# Autodesk Inventor assembly: Frame 1647030135921
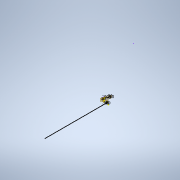
[picture p0: Inventor's stored thumbnail of the model, 180x180]
Saved by Autodesk Inventor 2022.2 (Build 262287010, 287A)
## iProperties
_FrameDoc: Frame Assembly
_Version: 25.0.0
Created: 2022-03-11
Part Number: Frame 1647030135921
Document SubType Name: Assembly
Designer: foriw
Mass: 6298.67 g
Surface Area: 9103.39 cm^2
Volume: 2238.81 cm^3
Density: 2.8134 g/cm^3
Author: foriw
## Documents named in this file (28)
- C:\Users\Finn Oriwohl\Documents\htx\1g g\BeerCart-CAD-Inventor\Workspaces\Workspace\beercart assembly - mekatronik\Frame\Frame 1647030135921.iam
- C:\Users\Finn Oriwohl\Documents\htx\1g g\BeerCart-CAD-Inventor\Workspaces\Workspace\beercart assembly - mekatronik\Frame\Skeleton 1647030135922.ipt
- C:\Users\Finn Oriwohl\Documents\htx\1g g\BeerCart-CAD-Inventor\Workspaces\Workspace\beercart assembly - mekatronik\Frame\ISO 12633-2 20x20x2 1647030639616.ipt
- C:\Users\Finn Oriwohl\Documents\htx\1g g\BeerCart-CAD-Inventor\Workspaces\Workspace\beercart assembly - mekatronik\Frame\ISO 12633-2 20x20x2 1647030639707.ipt
- C:\Users\Finn Oriwohl\Documents\htx\1g g\BeerCart-CAD-Inventor\Workspaces\Workspace\beercart assembly - mekatronik\Frame\ISO 12633-2 20x20x2 1647606177438.ipt
- C:\Users\Finn Oriwohl\Documents\htx\1g g\BeerCart-CAD-Inventor\Workspaces\Workspace\BackWheelMountingPlate.ipt
- C:\Users\Finn Oriwohl\Documents\htx\1g g\BeerCart-CAD-Inventor\Workspaces\Workspace\BackWheelMountingPlate_MIR_MIR.ipt
- C:\Users\Finn Oriwohl\Documents\htx\1g g\BeerCart-CAD-Inventor\Workspaces\Workspace\beercart assembly - mekatronik\Frame\ISO 12633-2 20x20x2 1648573909221.ipt
- C:\Users\Finn Oriwohl\Documents\htx\1g g\BeerCart-CAD-Inventor\Workspaces\Workspace\beercart assembly - mekatronik\Frame\ISO 12633-2 20x20x2 1648573975084.ipt
- C:\Users\Finn Oriwohl\Documents\htx\1g g\BeerCart-CAD-Inventor\Workspaces\Workspace\beercart assembly - mekatronik\Frame\ISO 12633-2 20x20x2 1648627088055.ipt
- C:\Users\Finn Oriwohl\Documents\htx\1g g\BeerCart-CAD-Inventor\Workspaces\Workspace\beercart assembly - mekatronik\Frame\ISO 12633-2 20x20x2 1648627088175.ipt
- C:\Users\Finn Oriwohl\Documents\htx\1g g\BeerCart-CAD-Inventor\Workspaces\Workspace\BackWheelMountingPlate_MIR4.ipt
- C:\Users\Finn Oriwohl\Documents\htx\1g g\BeerCart-CAD-Inventor\Workspaces\Workspace\beercart assembly - mekatronik\Frame\ISO 12633-2 20x20x2 1649085652950.ipt
- C:\Users\Finn Oriwohl\Documents\htx\1g g\BeerCart-CAD-Inventor\Workspaces\Workspace\beercart assembly - mekatronik\Frame\ISO 12633-2 20x20x2 1649085653040.ipt
- C:\Users\Finn Oriwohl\Documents\htx\1g g\BeerCart-CAD-Inventor\Workspaces\Workspace\backWheelNoMotor brake mount.ipt
- C:\Users\Finn Oriwohl\Documents\htx\1g g\BeerCart-CAD-Inventor\Workspaces\Workspace\beercart assembly - mekatronik\Frame\ISO 12633-2 20x20x2 1649154464355.ipt
- C:\Users\Finn Oriwohl\Documents\htx\1g g\BeerCart-CAD-Inventor\Workspaces\Workspace\BackWheelMotorMountSpacer.ipt
- C:\Users\Finn Oriwohl\Documents\htx\1g g\BeerCart-CAD-Inventor\Workspaces\Workspace\beercart assembly - mekatronik\Frame\FrontWheelFrameNew.iam
- C:\Users\Finn Oriwohl\Documents\htx\1g g\BeerCart-CAD-Inventor\Workspaces\Workspace\headset bearing.ipt
- C:\Users\Finn Oriwohl\Documents\htx\1g g\BeerCart-CAD-Inventor\Workspaces\Workspace\beercart assembly - mekatronik\Frame\ISO 12633-2 20x20x2 1650129877673.ipt
- C:\Users\Finn Oriwohl\Documents\htx\1g g\BeerCart-CAD-Inventor\Workspaces\Workspace\beercart assembly - mekatronik\Frame\ISO 12633-2 20x20x2 1650129879551.ipt
- C:\Users\Finn Oriwohl\Documents\htx\1g g\BeerCart-CAD-Inventor\Workspaces\Workspace\beercart assembly - mekatronik\Frame\ISO 12633-2 20x20x2 1650129879650.ipt
- C:\Users\Finn Oriwohl\Documents\htx\1g g\BeerCart-CAD-Inventor\Workspaces\Workspace\beercart assembly - mekatronik\Frame\ISO 12633-2 20x20x2 1650129879749.ipt
- C:\Users\Finn Oriwohl\Documents\htx\1g g\BeerCart-CAD-Inventor\Workspaces\Workspace\beercart assembly - mekatronik\Frame\ISO 12633-2 20x20x2 1650134807858.ipt
- C:\Users\Finn Oriwohl\Documents\htx\1g g\BeerCart-CAD-Inventor\Workspaces\Workspace\beercart assembly - mekatronik\Frame\plan1 .iam
- C:\Users\Finn Oriwohl\Documents\htx\1g g\BeerCart-CAD-Inventor\Workspaces\Workspace\beercart assembly - mekatronik\Frame\Plan 2 øverste.iam
- C:\Users\Finn Oriwohl\Documents\htx\1g g\BeerCart-CAD-Inventor\Workspaces\Workspace\beercart assembly - mekatronik\Frame\GlidelejrehusAssembly.iam
- C:\Users\Finn Oriwohl\Documents\htx\1g g\BeerCart-CAD-Inventor\Libraries\Content Center Files\en-US\ISO 4762(2)\ISO 4762 - M6 x 20ISO.ipt
## Components (31 placed, 23 different names)
1. Reference Skeleton
2. ISO 12633-2 20x20x2 - 250,13:1
3. ISO 12633-2 20x20x2 - 250,13:2
4. ISO 12633-2 20x20x2 - 123,73:2 — Mate:2, Mate:4, Mate:5
5. BackWheelMountingPlate:1 — Flush:6, Rotational:2, Rigid:1
6. BackWheelMountingPlate_MIR_MIR:1
7. ISO 12633-2 20x20x2 - 360,44:1
8. ISO 12633-2 20x20x2 - 105,43:1 — Flush:6, Rotational:2, Rigid:1
9. ISO 12633-2 20x20x2 - 107,97:1 — Flush:9, Flush:11, Flush:12, Flush:13, Rigid:2
10. ISO 12633-2 20x20x2 - 115.41:1
11. BackWheelMountingPlate_MIR4:1 — Flush:9, Rigid:2
12. ISO 12633-2 20x20x2 - 120.65:1 — Flush:14
13. ISO 12633-2 20x20x2 - 113,38:1 — Flush:10
14. backWheelNoMotor brake mount:1 — Flush:10, Flush:14
15. ISO 12633-2 20x20x2 - 105,43:1
16. BackWheelMotorMountSpacer:1 — Flush:11, Flush:12, Flush:13
17. FrontWheelFrameNew:1 [sub-assembly] — Insert:3, Insert:4
18. headset bearing:1 — Insert:3
19. ISO 12633-2 20x20x2 - 76,3:1
20. ISO 12633-2 20x20x2 - 85,41:1
21. ISO 12633-2 20x20x2 - 85,41:2 — Rigid:3
22. ISO 12633-2 20x20x2 - 76,3:2
23. ISO 12633-2 20x20x2 - 98,29:1
24. plan1 :1 [sub-assembly]
25. Plan 2 øverste:1 [sub-assembly]
26. GlidelejrehusAssembly:1 [sub-assembly] — Mate:20, Mate:21, Mate:22, Mate:23, Insert:4
27. GlidelejrehusAssembly:2 [sub-assembly] — Rigid:3, Mate:24, Mate:25, Mate:26, Mate:27
28. ISO 4762 M6 x 20:1 — Mate:20, Mate:21
29. ISO 4762 M6 x 20:2 — Mate:22, Mate:23
30. ISO 4762 M6 x 20:3 — Mate:24, Mate:25
31. ISO 4762 M6 x 20:4 — Mate:26, Mate:27
## Relationships (27: Mate 13, Flush 8, WeldJoint 3, Insert 2, RevoluteJoint 1)
- Mate:2: ISO 12633-2 20x20x2 - 123,73:2
- Mate:4: ISO 12633-2 20x20x2 - 123,73:2
- Mate:5: ISO 12633-2 20x20x2 - 123,73:2
- Flush:6: BackWheelMountingPlate:1 ↔ ISO 12633-2 20x20x2 - 105,43:1
- Rotational:2 [RevoluteJoint]: BackWheelMountingPlate:1 ↔ ISO 12633-2 20x20x2 - 105,43:1
- Flush:9: ISO 12633-2 20x20x2 - 107,97:1 ↔ BackWheelMountingPlate_MIR4:1
- Flush:10: ISO 12633-2 20x20x2 - 113,38:1 ↔ backWheelNoMotor brake mount:1
- Rigid:1 [WeldJoint]: BackWheelMountingPlate:1 ↔ ISO 12633-2 20x20x2 - 105,43:1
- Flush:11: ISO 12633-2 20x20x2 - 107,97:1 ↔ BackWheelMotorMountSpacer:1
- Flush:12: ISO 12633-2 20x20x2 - 107,97:1 ↔ BackWheelMotorMountSpacer:1
- Flush:13: ISO 12633-2 20x20x2 - 107,97:1 ↔ BackWheelMotorMountSpacer:1
- Flush:14: ISO 12633-2 20x20x2 - 120.65:1 ↔ backWheelNoMotor brake mount:1
- Insert:3: FrontWheelFrameNew:1 ↔ headset bearing:1
- Rigid:2 [WeldJoint]: ISO 12633-2 20x20x2 - 107,97:1 ↔ BackWheelMountingPlate_MIR4:1
- [Flush]: ISO 12633-2 20x20x2 - 85,41:1 ↔ GlidelejrehusAssembly:1
- [Mate]: FrontWheelFrameNew:1 ↔ GlidelejrehusAssembly:1
- [Mate]: ISO 12633-2 20x20x2 - 85,41:1 ↔ GlidelejrehusAssembly:1
- Rigid:3 [WeldJoint]: ISO 12633-2 20x20x2 - 85,41:2 ↔ GlidelejrehusAssembly:2
- Mate:20: GlidelejrehusAssembly:1 ↔ ISO 4762 M6 x 20:1
- Mate:21: GlidelejrehusAssembly:1 ↔ ISO 4762 M6 x 20:1
- Mate:22: GlidelejrehusAssembly:1 ↔ ISO 4762 M6 x 20:2
- Mate:23: GlidelejrehusAssembly:1 ↔ ISO 4762 M6 x 20:2
- Mate:24: GlidelejrehusAssembly:2 ↔ ISO 4762 M6 x 20:3
- Mate:25: GlidelejrehusAssembly:2 ↔ ISO 4762 M6 x 20:3
- Mate:26: GlidelejrehusAssembly:2 ↔ ISO 4762 M6 x 20:4
- Mate:27: GlidelejrehusAssembly:2 ↔ ISO 4762 M6 x 20:4
- Insert:4: FrontWheelFrameNew:1 ↔ GlidelejrehusAssembly:1
